# Autodesk Inventor assembly: main_idea
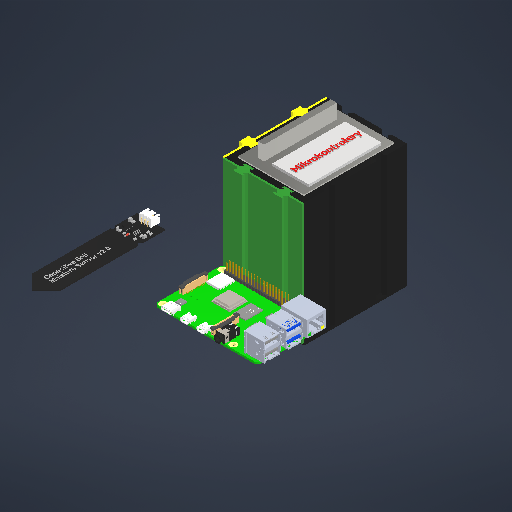
[picture p0: Inventor's stored thumbnail of the model, 512x512]
Saved by Autodesk Inventor 2027 (Build 310192060, 192F)
## iProperties
Created: 2026-06-08
Part Number: main_idea
Document SubType Name: Assembly
Designer: User
Author: User
## Documents named in this file (8)
- C:\Users\Duszy\Desktop\Shelf\main_idea.iam
- C:\Users\Duszy\Desktop\Shelf\connector.ipt
- C:\Users\Duszy\Desktop\Shelf\box.ipt
- C:\Users\Duszy\Desktop\Shelf\connector2.ipt
- C:\Users\Duszy\Desktop\Shelf\shelf.ipt
- C:\Users\Duszy\Desktop\Shelf\example of items\Moisture Sensor\Moisture Sensor.ipt
- C:\Users\Duszy\Desktop\Shelf\example of items\NUCLEO-F411RE\NUCLEO-F411RE.ipt
- C:\Users\Duszy\Desktop\Shelf\example of items\Raspberry Pi 4 Model B\Raspberry Pi 4 Model B.ipt
## Components (7 placed, 7 different names)
1. connector2:1 — Sztywne:2
2. box:1 — Sztywne:1, Sztywne:2, Walcowe:1
3. connector:1 — Sztywne:1
4. shelf:1 — Walcowe:1
5. Moisture Sensor:1
6. NUCLEO-F411RE:1
7. Raspberry Pi 4 Model B:1
## Relationships (3: WeldJoint 2, CylindricalJoint 1)
- Sztywne:1 [WeldJoint] (0.04 mm): box:1 ↔ connector:1
- Sztywne:2 [WeldJoint] (0.05 mm): connector2:1 ↔ box:1
- Walcowe:1 [CylindricalJoint]: box:1 ↔ shelf:1
